# Autodesk Inventor assembly: 6498K602 Pneumatic Cylinder Assembly
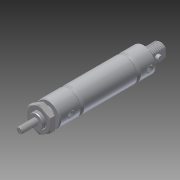
[picture p0: Inventor's stored thumbnail of the model, 180x180]
Saved by Autodesk Inventor 2014 SP1 (Build 180222100, 222)
## iProperties
Created: 2014-01-06
Part Number: 6498K602 Pneumatic Cylinder Assembly
Document SubType Name: Assembly
Designer: Moses
Mass: 67.9237 g
Surface Area: 107.189 cm^2
Volume: 20.2084 cm^3
Density: 3.36116 g/cm^3
Author: Moses
## Documents named in this file (4)
- C:\Users\Arpan\Documents\GitHub\2014buildCAD\Shooter\6498K602 Pneumatic Cylinder Assembly.iam
- C:\Users\Arpan\Documents\GitHub\2014buildCAD\Shooter\6498K602 Body.ipt
- C:\Users\Arpan\Documents\GitHub\2014buildCAD\Shooter\6498K602 Rod.ipt
- C:\Users\Arpan\Documents\GitHub\2014buildCAD\Shooter\6498K602 Nut.ipt
## Components (3 placed, 3 different names)
1. 6498K602 Body:1 — Mate:1, Flush:1, Insert:1
2. 6498K602 Rod:1 — Mate:1, Flush:1
3. 6498K602 Nut:1 — Insert:1
## Relationships (3: Mate 1, Flush 1, Insert 1)
- Mate:1: 6498K602 Body:1 ↔ 6498K602 Rod:1
- Flush:1 (-12.7 mm): 6498K602 Body:1 ↔ 6498K602 Rod:1
- Insert:1 (3.175 mm): 6498K602 Body:1 ↔ 6498K602 Nut:1
